# Autodesk Inventor assembly: Pressure Vessel, Global Assembly
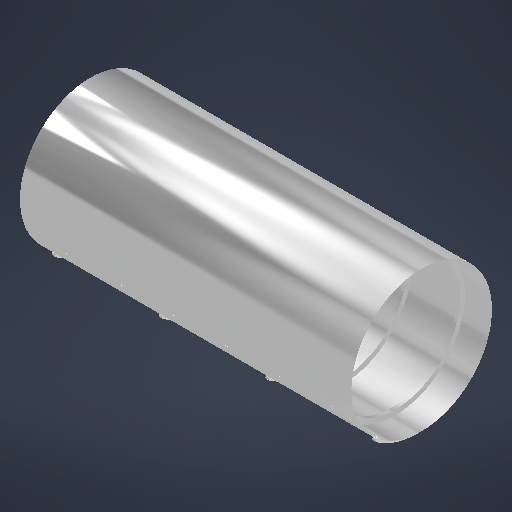
[picture p0: Inventor's stored thumbnail of the model, 512x512]
Saved by Autodesk Inventor 2026 (Build 300175000, 175)
## iProperties
Created: 2025-10-25
Part Number: Pressure Vessel, Global Assembly
Document SubType Name: Assembly
Designer: Brandon Portillo
Mass: 2.22051e+06 g
Surface Area: 3.10148e+06 cm^2
Volume: 890936 cm^3
Density: 2.49233 g/cm^3
Author: Brandon Portillo
## iProperties of the stored document MemberDocs/xRd31mju1Fs0ltyt4Lrp1urqlEg
Created: 2025-10-25
Part Number: Pressure Vessel, Global Assembly
Document SubType Name: Assembly
Designer: Brandon Portillo
Mass: 2.22051e+06 g
Surface Area: 3.10148e+06 cm^2
Volume: 890936 cm^3
Density: 2.49233 g/cm^3
Author: Brandon Portillo
## Documents named in this file (23)
- C:\Users\anarc\GitHub\TSGC-NASA_Senior_Design\CAD\Pressure Vessel\Pressure Vessel, Global Assembly.iam
- C:\Users\anarc\GitHub\TSGC-NASA_Senior_Design\CAD\Pressure Vessel\Pressure Vessel, Single Part.ipt
- C:\Users\anarc\GitHub\TSGC-NASA_Senior_Design\CAD\Pressure Vessel\Saddle.ipt
- C:\Users\anarc\GitHub\TSGC-NASA_Senior_Design\CAD\Pressure Vessel\Doubler Plate, Bolted and Welded.ipt
- C:\Users\anarc\GitHub\TSGC-NASA_Senior_Design\CAD\Pressure Vessel\Support Ring, L-Section.ipt
- C:\Users\anarc\GitHub\TSGC-NASA_Senior_Design\CAD\Pressure Vessel\Pressure Vessel, Global Assembly\AIP\FEA\f8hakl7hc.fins
- C:\Users\anarc\GitHub\TSGC-NASA_Senior_Design\CAD\Pressure Vessel\Pressure Vessel, Global Assembly\AIP\FEA\f8hakl7hc.fsat
- C:\Users\anarc\GitHub\TSGC-NASA_Senior_Design\CAD\Pressure Vessel\Pressure Vessel, Global Assembly\AIP\FEA\f8hakl7hc.ftes
- C:\Users\anarc\GitHub\TSGC-NASA_Senior_Design\CAD\Pressure Vessel\Pressure Vessel, Global Assembly\AIP\FEA\f8hakl7hc.fwiz
- C:\Users\anarc\GitHub\TSGC-NASA_Senior_Design\CAD\Pressure Vessel\Pressure Vessel, Global Assembly\AIP\FEA\f8hakl7i8.fmsh
- C:\Users\anarc\GitHub\TSGC-NASA_Senior_Design\CAD\Pressure Vessel\Pressure Vessel, Global Assembly\AIP\FEA\f8hakl7i9.fres
- C:\Users\anarc\GitHub\TSGC-NASA_Senior_Design\CAD\Pressure Vessel\Pressure Vessel, Global Assembly\AIP\FEA\f8iii2myo.fins
- C:\Users\anarc\GitHub\TSGC-NASA_Senior_Design\CAD\Pressure Vessel\Pressure Vessel, Global Assembly\AIP\FEA\f8iii2myo.fsat
- C:\Users\anarc\GitHub\TSGC-NASA_Senior_Design\CAD\Pressure Vessel\Pressure Vessel, Global Assembly\AIP\FEA\f8iii2myo.ftes
- C:\Users\anarc\GitHub\TSGC-NASA_Senior_Design\CAD\Pressure Vessel\Pressure Vessel, Global Assembly\AIP\FEA\f8iii2myo.fwiz
- C:\Users\anarc\GitHub\TSGC-NASA_Senior_Design\CAD\Pressure Vessel\Pressure Vessel, Global Assembly\AIP\FEA\f8iii2n40.fmsh
- C:\Users\anarc\GitHub\TSGC-NASA_Senior_Design\CAD\Pressure Vessel\Pressure Vessel, Global Assembly\AIP\FEA\f8iii2n4w.fres
- C:\Users\anarc\GitHub\TSGC-NASA_Senior_Design\CAD\Pressure Vessel\Pressure Vessel, Global Assembly\AIP\FEA\f8iu11i74.fins
- C:\Users\anarc\GitHub\TSGC-NASA_Senior_Design\CAD\Pressure Vessel\Pressure Vessel, Global Assembly\AIP\FEA\f8iu11i74.fsat
- C:\Users\anarc\GitHub\TSGC-NASA_Senior_Design\CAD\Pressure Vessel\Pressure Vessel, Global Assembly\AIP\FEA\f8iu11i74.ftes
- C:\Users\anarc\GitHub\TSGC-NASA_Senior_Design\CAD\Pressure Vessel\Pressure Vessel, Global Assembly\AIP\FEA\f8iu11i74.fwiz
- C:\Users\anarc\GitHub\TSGC-NASA_Senior_Design\CAD\Pressure Vessel\Pressure Vessel, Global Assembly\AIP\FEA\f8iu11iao.fmsh
- C:\Users\anarc\GitHub\TSGC-NASA_Senior_Design\CAD\Pressure Vessel\Pressure Vessel, Global Assembly\AIP\FEA\f8iu11iap.fres
## Components (29 placed, 4 different names)
1. Pressure Vessel, Single Part:1 — Mate:8, Flush:15, Tangent:1, Angle:1, Mate:10, Angle:2, Mate:11, Flush:16
2. Saddle:1 — Mate:8, Flush:15
3. Saddle:2
4. Saddle:3
5. Saddle:4
6. Support Ring, L-Section:1 — Mate:11, Flush:16
7. Support Ring, L-Section:2
8. Support Ring, L-Section:3
9. Support Ring, L-Section:4
10. Support Ring, L-Section:5
11. Support Ring, L-Section:6
12. Doubler Plate, Bolted and Welded:1 — Tangent:1, Angle:1, Mate:10, Angle:2
13. Doubler Plate, Bolted and Welded:2
14. Doubler Plate, Bolted and Welded:3
15. Doubler Plate, Bolted and Welded:4
16. Doubler Plate, Bolted and Welded:5
17. Doubler Plate, Bolted and Welded:6
18. Doubler Plate, Bolted and Welded:7
19. Doubler Plate, Bolted and Welded:8
20. Doubler Plate, Bolted and Welded:9
21. Doubler Plate, Bolted and Welded:10
22. Doubler Plate, Bolted and Welded:11
23. Doubler Plate, Bolted and Welded:12
24. Doubler Plate, Bolted and Welded:13
25. Doubler Plate, Bolted and Welded:14
26. Doubler Plate, Bolted and Welded:15
27. Doubler Plate, Bolted and Welded:16
28. Doubler Plate, Bolted and Welded:17
29. Doubler Plate, Bolted and Welded:18
## Component patterns: (4 elements, first: Saddle:1), (6 elements, first: Support Ring, L-Section:1), (3 elements, first: Doubler Plate, Bolted and Welded:1), Component Pattern 7:2 (3 elements), Component Pattern 7:3 (3 elements), Component Pattern 7:4 (3 elements), Component Pattern 7:5 (3 elements), Component Pattern 7:6 (3 elements)
## Relationships (8: Mate 3, Flush 2, Angle 2, Tangent 1)
- Mate:8: Pressure Vessel, Single Part:1 ↔ Saddle:1
- Flush:15 (100 mm): Pressure Vessel, Single Part:1 ↔ Saddle:1
- Tangent:1: Pressure Vessel, Single Part:1 ↔ Doubler Plate, Bolted and Welded:1
- Angle:1 (0 deg): Pressure Vessel, Single Part:1 ↔ Doubler Plate, Bolted and Welded:1
- Mate:10 (750 mm): Pressure Vessel, Single Part:1 ↔ Doubler Plate, Bolted and Welded:1
- Angle:2 (120 deg): Pressure Vessel, Single Part:1 ↔ Doubler Plate, Bolted and Welded:1
- Mate:11: Pressure Vessel, Single Part:1 ↔ Support Ring, L-Section:1
- Flush:16 (800 mm): Pressure Vessel, Single Part:1 ↔ Support Ring, L-Section:1
## Named parameters: sa_0 = 0, sa_1 = -981, sa_2 = 0, sa_3 = 5886
note: some values were not read from the file. Shown as the stored number, unit unknown: "sa_0", "sa_1", "sa_2", "sa_3".
